# Autodesk Inventor assembly: Assembly1
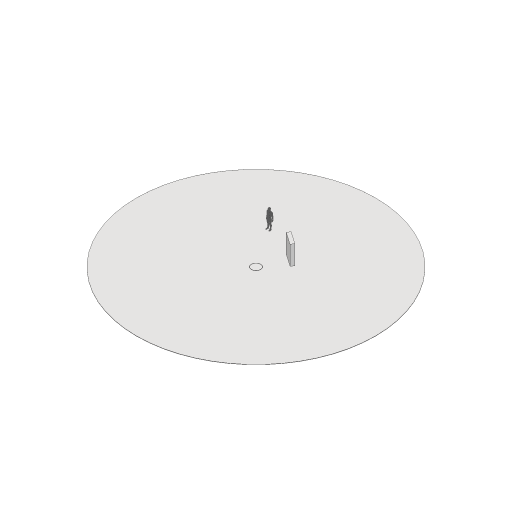
[picture p0: Inventor's stored thumbnail of the model, 512x512]
Saved by Autodesk Inventor 2023 (Build 270158000, 158)
## iProperties
Created: 2022-08-15
Part Number: Assembly1
Document SubType Name: Assembly
Designer: Derm
Author: Derm
## Documents named in this file (4)
- C:\Users\Derm\vaRLnt\v3\perspective_shift\figures\Assembly1.iam
- C:\Users\Derm\vaRLnt\v3\perspective_shift\figures\world.ipt
- C:\Users\Derm\vaRLnt\v3\perspective_shift\training_data\Imported Components\car1\car1.ipt
- C:\Users\Derm\vaRLnt\v3\perspective_shift\training_data\Imported Components\dummy\dummy.ipt
## Components (3 placed, 3 different names)
1. world:1 — Flush:1
2. car1:1
3. dummy:1
## Relationships (1: Flush 1)
- Flush:1: world:1
